# Autodesk Inventor assembly: Assembly1
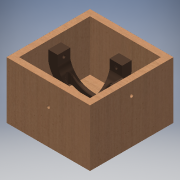
[picture p0: Inventor's stored thumbnail of the model, 180x180]
Saved by Autodesk Inventor 2017 (Build 210142000, 142)
## iProperties
Created: 2017-01-26
Part Number: Assembly1
Document SubType Name: Assembly
Designer: aribu
Author: aribu
## Documents named in this file (3)
- C:\Users\aribu\Documents\Assembly1.iam
- C:\Users\aribu\Documents\Box.ipt
- C:\Users\aribu\Documents\Arms1.ipt
## Components (3 placed, 2 different names)
1. Box:1 — Rotational:1, Rotational:2
2. Arms1:1 — Rotational:1
3. Arms1:2 — Rotational:2
## Relationships (2: RevoluteJoint 2)
- Rotational:1 [RevoluteJoint]: Box:1 ↔ Arms1:1
- Rotational:2 [RevoluteJoint]: Box:1 ↔ Arms1:2
